# Autodesk Inventor assembly: Drivetrain_Assembly_V1
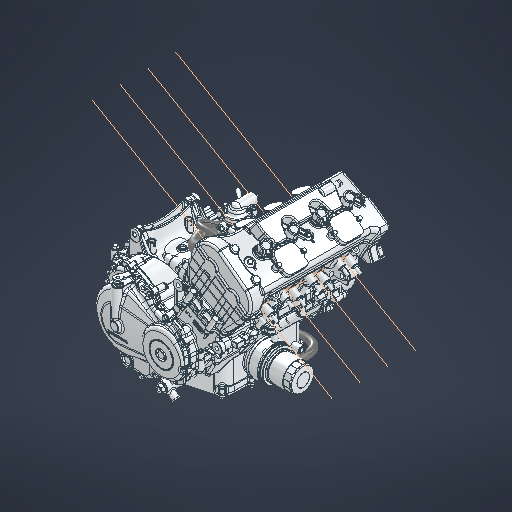
[picture p0: Inventor's stored thumbnail of the model, 512x512]
Saved by Autodesk Inventor 2026.1 (Build 301233000, 233)
## iProperties
Created: 2026-07-20
Part Number: Drivetrain_Assembly_V1
Document SubType Name: Assembly
Designer: share
Author: share
## Documents named in this file (2)
- C:\Users\share\OneDrive\Documents\Personal Projects\GOGO Kart\CAD\GOGO_KART_FSAE\Drivetrain\Drivetrain_Assembly_V1.iam
- C:\Users\share\OneDrive\Documents\Personal Projects\GOGO Kart\CAD\GOGO_KART_FSAE\Drivetrain\honda-cbr600-f4i-engine-1.snapshot.3\Honda CBR600 F4i\Honda CBR600 F4i\Honda CBR600 F4i.ipt
## Components (1 placed, 1 different names)
1. Honda CBR600 F4i:1 — Flush:1, Mate:1, Flush:2, Mate:3, Mate:4, Mate:5, Mate:6
## Relationships (9: Mate 7, Flush 2)
- Flush:1: Honda CBR600 F4i:1
- Mate:1: Honda CBR600 F4i:1
- Flush:2: Honda CBR600 F4i:1
- Mate:3: Honda CBR600 F4i:1
- Mate:4: Honda CBR600 F4i:1
- Mate:5: Honda CBR600 F4i:1
- Mate:6: Honda CBR600 F4i:1
- Mate:7
- Mate:8
